# Autodesk Inventor assembly: OdomHorizontal
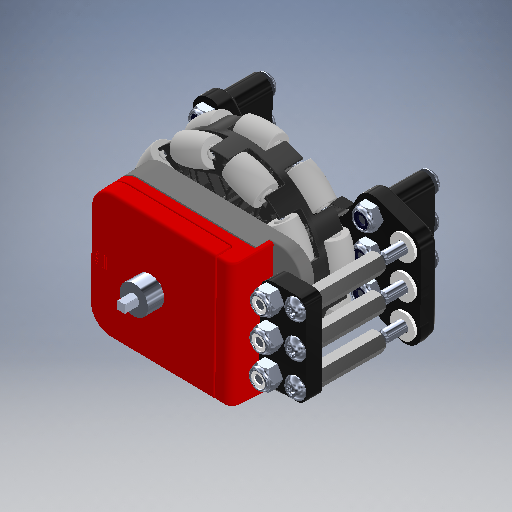
[picture p0: Inventor's stored thumbnail of the model, 512x512]
Saved by Autodesk Inventor 2026.1 (Build 301233000, 233)
## iProperties
Created: 2025-10-06
Part Number: OdomHorizontal
Document SubType Name: Assembly
Designer: Teddy
Author: Teddy
## Documents named in this file (27)
- C:\Users\Teddy\Desktop\VexCAD\15InVEX\OdomHorizontal.iam
- C:\Users\Teddy\Desktop\VexCAD\VEX-CAD-Inventor\Motion\Wheels\Omni Wheel\2.75 Omni AS, No Insert.iam
- C:\Users\Teddy\Desktop\VexCAD\VEX-CAD-Inventor\Motion\Wheels\Omni Wheel.iam
- C:\Users\Teddy\Desktop\VexCAD\VEX-CAD-Inventor\Electronics\Sensors\Optical Shaft Encoder.ipt
- C:\Users\Teddy\Desktop\VexCAD\VEX-CAD-Inventor\Motion\Spacers\Spacer Nylon .500 OD.ipt
- C:\Users\Teddy\Desktop\VexCAD\VEX-CAD-Inventor\Motion\Spacers\Spacer Nylon .500 OD\NSpacer White .500 OD x .375.ipt
- C:\Users\Teddy\Desktop\VexCAD\15InVEX\OdomPods.ipt
- C:\Users\Teddy\Desktop\VexCAD\15InVEX\OdomPodPart2.ipt
- C:\Users\Teddy\Desktop\VexCAD\VEX-CAD-Inventor\Motion\Shaft LS\Bearing Flat.ipt
- C:\Users\Teddy\Desktop\VexCAD\VEX-CAD-Inventor\Structure\Standoff\Standoff 1.00.ipt
- C:\Users\Teddy\Desktop\VexCAD\VEX-CAD-Inventor\Structure\Standoff.ipt
- C:\Users\Teddy\Desktop\VexCAD\VEX-CAD-Inventor\Motion\Spacers\Washer Teflon\TWasher .375 OD x .04000.ipt
- C:\Users\Teddy\Desktop\VexCAD\VEX-CAD-Inventor\Motion\Spacers\Washer Teflon.ipt
- C:\Users\Teddy\Desktop\VexCAD\VEX-CAD-Inventor\Structure\Hardware\Screw Steel - Star\SScrew Star Smooth .750.ipt
- C:\Users\Teddy\Desktop\VexCAD\VEX-CAD-Inventor\Structure\Hardware\Screw Steel - Star.ipt
- C:\Users\Teddy\Desktop\VexCAD\VEX-CAD-Inventor\Structure\Hardware\Nut Nylock.ipt
- C:\Users\Teddy\Desktop\VexCAD\VEX-CAD-Inventor\Motion\Shaft LS\Shaft LS Capped\Shaft LS Capped 3.0.ipt
- C:\Users\Teddy\Desktop\VexCAD\VEX-CAD-Inventor\Motion\Shaft LS\Shaft LS Capped.ipt
- C:\Users\Teddy\Desktop\VexCAD\VEX-CAD-Inventor\Motion\Shaft LS\Shaft Collar Metal\Shaft Collar No Screw.iam
- C:\Users\Teddy\Desktop\VexCAD\VEX-CAD-Inventor\Motion\Shaft LS\Shaft Collar Metal.iam
- C:\Users\Teddy\Desktop\VexCAD\VEX-CAD-Inventor\Structure\Hardware\Screw Steel - Star\SScrew Star Smooth .625.ipt
- C:\Users\Teddy\Desktop\VexCAD\VEX-CAD-Inventor\Structure\Hardware\Screw Steel - Star\SScrew Star Smooth .500.ipt
- C:\Users\Teddy\Desktop\VexCAD\VEX-CAD-Inventor\Motion\Spacers\Spacer Nylon .500 OD\NSpacer Black .500 OD x .125.ipt
- C:\Users\Teddy\Desktop\VexCAD\VEX-CAD-Inventor\Structure\Hardware\Nut Thin Nylock.ipt
- C:\Users\Teddy\Desktop\VexCAD\VEX-CAD-Inventor\Structure\Hardware\Screw Steel - Star\SScrew Star Smooth 1.000.ipt
- C:\Users\Teddy\Desktop\VexCAD\VEX-CAD-Inventor\Motion\Spacers\Spacer Nylon .375 OD\NSpacer .375 OD x .250.ipt
- C:\Users\Teddy\Desktop\VexCAD\VEX-CAD-Inventor\Motion\Spacers\Spacer Nylon .375 OD.ipt
## Components (47 placed, 18 different names)
1. 2.75 Omni AS, No Insert:1 [sub-assembly] — Insert:1, Insert:54
2. Optical Shaft Encoder:1 — Insert:2, Flush:1, Flush:2, Insert:20, Insert:24, Insert:25, Insert:26
3. NSpacer White .500 OD x .375:1 — Insert:1, Insert:2
4. OdomPods:1 — Flush:1, Flush:2, Insert:6, Insert:7, Insert:8, Insert:27, Insert:28, Insert:29, Insert:30, Insert:31, Insert:32
5. OdomPodPart2:1 — Insert:4, Insert:5, Insert:17, Insert:18, Insert:37, Insert:38, Insert:39, Insert:40, Insert:41, Insert:42, Insert:43, Insert:44, Insert:45, Insert:46, Insert:47, Insert:48, Insert:49, Insert:50, Insert:51, Insert:53
6. Bearing Flat:1 — Insert:4, Insert:5, Insert:15, Insert:16, Insert:19
7. Standoff 1.00:1 — Insert:6
8. Standoff 1.00:2 — Insert:7
9. Standoff 1.00:3 — Insert:8
10. TWasher .375 OD x .04000:1 — Insert:35
11. TWasher .375 OD x .04000:2 — Insert:36
12. TWasher .375 OD x .04000:3 — Insert:34
13. SScrew Star Smooth .750:1 — Insert:15
14. SScrew Star Smooth .750:2 — Insert:16
15. Nut Nylock:1 — Insert:18
16. Nut Nylock:2 — Insert:17
17. Shaft LS Capped 3.0:1 — Insert:19
18. Shaft Collar No Screw:1 [sub-assembly] — Insert:20
19. SScrew Star Smooth .625:4 — Insert:24
20. SScrew Star Smooth .625:5 — Insert:25
21. SScrew Star Smooth .625:8 — Insert:26
22. SScrew Star Smooth .500:9 — Insert:27
23. SScrew Star Smooth .500:10 — Insert:28
24. SScrew Star Smooth .500:11 — Insert:29
25. Nut Nylock:3 — Insert:30
26. Nut Nylock:4 — Insert:31
27. Nut Nylock:5 — Insert:32
28. NSpacer Black .500 OD x .125:6 — Insert:52, Insert:54
29. NSpacer Black .500 OD x .125:7 — Insert:34
30. NSpacer Black .500 OD x .125:8 — Insert:35
31. NSpacer Black .500 OD x .125:9 — Insert:36
32. SScrew Star Smooth .500:12 — Insert:37
33. SScrew Star Smooth .500:13 — Insert:38
34. SScrew Star Smooth .500:14 — Insert:39
35. Nut Thin Nylock:1 — Insert:44
36. Nut Thin Nylock:2 — Insert:45
37. Nut Thin Nylock:3 — Insert:43
38. Nut Thin Nylock:4 — Insert:40
39. Nut Thin Nylock:5 — Insert:41
40. Nut Thin Nylock:6 — Insert:42
41. SScrew Star Smooth 1.000:15 — Insert:46
42. SScrew Star Smooth 1.000:16 — Insert:47
43. SScrew Star Smooth 1.000:17 — Insert:48
44. SScrew Star Smooth 1.000:18 — Insert:49
45. SScrew Star Smooth 1.000:19 — Insert:50
46. SScrew Star Smooth 1.000:20 — Insert:51
47. NSpacer .375 OD x .250:1 — Insert:52, Insert:53
## Relationships (45: Insert 43, Flush 2)
- Insert:1: 2.75 Omni AS, No Insert:1 ↔ NSpacer White .500 OD x .375:1
- Insert:2 (0.508 mm): Optical Shaft Encoder:1 ↔ NSpacer White .500 OD x .375:1
- Flush:1: Optical Shaft Encoder:1 ↔ OdomPods:1
- Flush:2: Optical Shaft Encoder:1 ↔ OdomPods:1
- Insert:4: OdomPodPart2:1 ↔ Bearing Flat:1
- Insert:5: OdomPodPart2:1 ↔ Bearing Flat:1
- Insert:6: OdomPods:1 ↔ Standoff 1.00:1
- Insert:7: OdomPods:1 ↔ Standoff 1.00:2
- Insert:8: OdomPods:1 ↔ Standoff 1.00:3
- Insert:15: Bearing Flat:1 ↔ SScrew Star Smooth .750:1
- Insert:16: Bearing Flat:1 ↔ SScrew Star Smooth .750:2
- Insert:17: OdomPodPart2:1 ↔ Nut Nylock:2
- Insert:18: OdomPodPart2:1 ↔ Nut Nylock:1
- Insert:19: Bearing Flat:1 ↔ Shaft LS Capped 3.0:1
- Insert:20 (0.635 mm): Optical Shaft Encoder:1 ↔ Shaft Collar No Screw:1
- Insert:24: Optical Shaft Encoder:1 ↔ SScrew Star Smooth .625:4
- Insert:25: Optical Shaft Encoder:1 ↔ SScrew Star Smooth .625:5
- Insert:26: Optical Shaft Encoder:1 ↔ SScrew Star Smooth .625:8
- Insert:27: OdomPods:1 ↔ SScrew Star Smooth .500:9
- Insert:28: OdomPods:1 ↔ SScrew Star Smooth .500:10
- Insert:29: OdomPods:1 ↔ SScrew Star Smooth .500:11
- Insert:30: OdomPods:1 ↔ Nut Nylock:3
- Insert:31: OdomPods:1 ↔ Nut Nylock:4
- Insert:32: OdomPods:1 ↔ Nut Nylock:5
- Insert:34: TWasher .375 OD x .04000:3 ↔ NSpacer Black .500 OD x .125:7
- Insert:35: TWasher .375 OD x .04000:1 ↔ NSpacer Black .500 OD x .125:8
- Insert:36: TWasher .375 OD x .04000:2 ↔ NSpacer Black .500 OD x .125:9
- Insert:37: OdomPodPart2:1 ↔ SScrew Star Smooth .500:12
- Insert:38: OdomPodPart2:1 ↔ SScrew Star Smooth .500:13
- Insert:39: OdomPodPart2:1 ↔ SScrew Star Smooth .500:14
- Insert:40: OdomPodPart2:1 ↔ Nut Thin Nylock:4
- Insert:41: OdomPodPart2:1 ↔ Nut Thin Nylock:5
- Insert:42: OdomPodPart2:1 ↔ Nut Thin Nylock:6
- Insert:43: OdomPodPart2:1 ↔ Nut Thin Nylock:3
- Insert:44: OdomPodPart2:1 ↔ Nut Thin Nylock:1
- Insert:45: OdomPodPart2:1 ↔ Nut Thin Nylock:2
- Insert:46 (1.27 mm): OdomPodPart2:1 ↔ SScrew Star Smooth 1.000:15
- Insert:47 (1.27 mm): OdomPodPart2:1 ↔ SScrew Star Smooth 1.000:16
- Insert:48 (1.27 mm): OdomPodPart2:1 ↔ SScrew Star Smooth 1.000:17
- Insert:49 (1.27 mm): OdomPodPart2:1 ↔ SScrew Star Smooth 1.000:18
- Insert:50 (1.27 mm): OdomPodPart2:1 ↔ SScrew Star Smooth 1.000:19
- Insert:51 (1.27 mm): OdomPodPart2:1 ↔ SScrew Star Smooth 1.000:20
- Insert:52: NSpacer Black .500 OD x .125:6 ↔ NSpacer .375 OD x .250:1
- Insert:53: OdomPodPart2:1 ↔ NSpacer .375 OD x .250:1
- Insert:54: 2.75 Omni AS, No Insert:1 ↔ NSpacer Black .500 OD x .125:6
